# Autodesk Inventor assembly: 30mm Fan
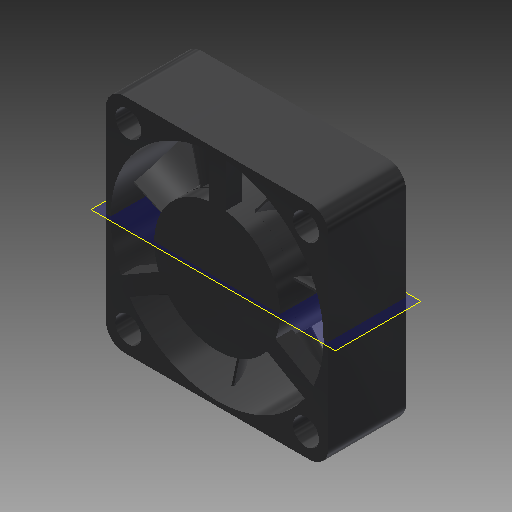
[picture p0: Inventor's stored thumbnail of the model, 512x512]
Saved by Autodesk Inventor 2018 (Build 220112000, 112)
## iProperties
Created: 2015-12-17
Part Number: 30mm Fan
Document SubType Name: Assembly
Designer: Jasper
Title: /vol/tmp/translate-1970156840469106288/56733729e4b0e545db4b6a25.step
## Documents named in this file (3)
- D:\Jasper's Stuff\git_WSL\MEME_MACHINE\CAD\Vitamins\30mm Fan.iam
- D:\Jasper's Stuff\git_WSL\MEME_MACHINE\CAD\Vitamins\30mm Fan Case.ipt
- D:\Jasper's Stuff\git_WSL\MEME_MACHINE\CAD\Vitamins\30mm Fan Blade.ipt
## Components (2 placed, 2 different names)
1. 30mm Fan Case — Mate:1, Flush:1
2. 30mm Fan Blade — Mate:1, Flush:1
## Relationships (2: Mate 1, Flush 1)
- Mate:1: 30mm Fan Case ↔ 30mm Fan Blade
- Flush:1: 30mm Fan Case ↔ 30mm Fan Blade
